# Autodesk Inventor assembly: Assembly Light Stack
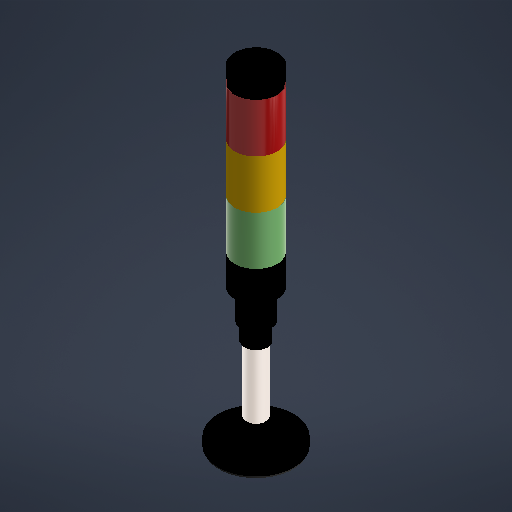
[picture p0: Inventor's stored thumbnail of the model, 512x512]
Saved by Autodesk Inventor 2027 (Build 310192000, 192)
## iProperties
Created: 2020-05-28
Part Number: Assembly Light Stack
Document SubType Name: Assembly
Designer: Sid
Author: Sid
## iProperties of the stored document MemberDocs/xAaaaqbcaAaaaaaaaAaaaqxjcCb
Created: 2020-05-28
Part Number: Assembly Light Stack
Document SubType Name: Assembly
Designer: Sid
Author: Sid
## Documents named in this file (5)
- C:\Users\ratik\OneDrive\Personal Folder\00_Startup\01_Mectosys_Prototype\01_Prototype\01_Mechanical\3D file\07_Comp\led-stack-light-indicator-signal-1.snapshot.3\Stack Light\Assembly Light Stack.iam
- C:\Users\ratik\OneDrive\Personal Folder\00_Startup\01_Mectosys_Prototype\01_Prototype\01_Mechanical\3D file\07_Comp\led-stack-light-indicator-signal-1.snapshot.3\Stack Light\Light Stack.ipt
- C:\Users\ratik\OneDrive\Personal Folder\00_Startup\01_Mectosys_Prototype\01_Prototype\01_Mechanical\3D file\07_Comp\led-stack-light-indicator-signal-1.snapshot.3\Stack Light\Connecting Rod.ipt
- C:\Users\ratik\OneDrive\Personal Folder\00_Startup\01_Mectosys_Prototype\01_Prototype\01_Mechanical\3D file\07_Comp\led-stack-light-indicator-signal-1.snapshot.3\Stack Light\Base.ipt
- C:\Users\ratik\OneDrive\Personal Folder\00_Startup\01_Mectosys_Prototype\01_Prototype\01_Mechanical\3D file\07_Comp\led-stack-light-indicator-signal-1.snapshot.3\Stack Light\Black Rubber Pad Bottom.ipt
## Components (4 placed, 4 different names)
1. Light Stack:1 — Cylindrical:1
2. Connecting Rod:1 — Cylindrical:1, Rotational:1
3. Base:1 — Rotational:1, Rotational:2
4. Black Rubber Pad Bottom:1 — Rotational:2
## Relationships (3: RevoluteJoint 2, CylindricalJoint 1)
- Cylindrical:1: Light Stack:1 ↔ Connecting Rod:1
- Rotational:1 [RevoluteJoint]: Connecting Rod:1 ↔ Base:1
- Rotational:2 [RevoluteJoint]: Base:1 ↔ Black Rubber Pad Bottom:1
